# Autodesk Inventor assembly: kitchen
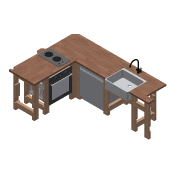
[picture p0: Inventor's stored thumbnail of the model, 180x180]
Saved by Autodesk Inventor 2018 (Build 220112000, 112)
## iProperties
Created: 2017-12-11
Part Number: kitchen
Document SubType Name: Assembly
Designer: sawaiz
Author: sawaiz
## Documents named in this file (12)
- C:\Users\sawaiz\OneDrive\personal\berlin\Move\larkspur\kitchen\kitchen.iam
- C:\Users\sawaiz\OneDrive\personal\berlin\Move\larkspur\kitchen\countertopSink.ipt
- C:\Users\sawaiz\OneDrive\personal\berlin\Move\larkspur\kitchen\Sink 63220001.ipt
- C:\Users\sawaiz\OneDrive\personal\berlin\Move\larkspur\kitchen\mieleWT946.ipt
- C:\Users\sawaiz\OneDrive\personal\berlin\Move\larkspur\kitchen\frameVertical.ipt
- C:\Users\sawaiz\OneDrive\personal\berlin\Move\larkspur\kitchen\frameSides.iam
- C:\Users\sawaiz\OneDrive\personal\berlin\Move\larkspur\kitchen\stoveCountertop.ipt
- C:\Users\sawaiz\OneDrive\personal\berlin\Move\larkspur\kitchen\Samsung BF641FGB.ipt
- C:\Users\sawaiz\OneDrive\personal\berlin\Move\larkspur\kitchen\Cooktop.ipt
- C:\Users\sawaiz\OneDrive\personal\berlin\Move\larkspur\kitchen\sink mixture DND assembly - sink mixture DND-1.ipt
- C:\Users\sawaiz\OneDrive\personal\berlin\Move\larkspur\kitchen\horizontalUnderSink.ipt
- C:\Users\sawaiz\OneDrive\personal\berlin\Move\larkspur\kitchen\kitchen.xlsx
## Components (15 placed, 10 different names)
1. countertopSink:1 — Flush:1, Mate:1, Mate:2, Mate:3, Flush:3, Mate:7, Flush:15, Mate:8, Flush:23, Flush:24, Mate:12, Flush:26, Mate:13, Flush:34, Mate:14, Mate:25
2. Sink 63220001:1 — Flush:1, Mate:1, Mate:2
3. mieleWT946:1 — Mate:3, Flush:3, Flush:16, Mate:9, Flush:33
4. frameVertical:5 — Mate:7, Flush:15, Flush:25
5. frameSides:1 [sub-assembly] — Flush:17, Flush:20, Flush:23, Flush:25
6. frameSides:2 [sub-assembly] — Flush:16, Flush:17, Flush:21, Mate:9, Flush:24, Flush:38, Flush:39
7. frameSides:4 [sub-assembly] — Flush:20, Flush:21, Mate:8, Mate:11, Angle:1, Flush:33
8. frameSides:5 [sub-assembly] — Mate:11, Angle:1, Mate:12, Flush:26, Mate:20, Flush:35
9. frameSides:7 [sub-assembly] — Mate:18, Mate:21, Mate:22, Mate:23, Flush:35, Flush:36
10. stoveCountertop:1 — Mate:13, Flush:34, Mate:14, Mate:19, Angle:2, Mate:23, Mate:24, Flush:37
11. Samsung BF641FGB:1 — Mate:18, Mate:20, Mate:21, Mate:22
12. Cooktop:1 — Mate:19, Angle:2
13. frameSides:8 [sub-assembly] — Flush:36, Mate:24, Flush:37
14. sink mixture DND assembly - sink mixture DND-1:1 — Mate:25
15. horizontalUnderSink:1 — Flush:38, Flush:39
## Relationships (38: Flush 18, Mate 18, Angle 2)
- Flush:1: countertopSink:1 ↔ Sink 63220001:1
- Mate:1: countertopSink:1 ↔ Sink 63220001:1
- Mate:2 (2.5 mm): countertopSink:1 ↔ Sink 63220001:1
- Mate:3: countertopSink:1 ↔ mieleWT946:1
- Flush:3 (50 mm): countertopSink:1 ↔ mieleWT946:1
- Mate:7: countertopSink:1 ↔ frameVertical:5
- Flush:15 (50 mm): countertopSink:1 ↔ frameVertical:5
- Flush:16: mieleWT946:1 ↔ frameSides:2
- Flush:17: frameSides:1 ↔ frameSides:2
- Flush:20: frameSides:1 ↔ frameSides:4
- Flush:21: frameSides:2 ↔ frameSides:4
- Mate:8: countertopSink:1 ↔ frameSides:4
- Mate:9 (2.5 mm): mieleWT946:1 ↔ frameSides:2
- Flush:23: countertopSink:1 ↔ frameSides:1
- Flush:24: countertopSink:1 ↔ frameSides:2
- Mate:11: frameSides:4 ↔ frameSides:5
- Angle:1 (270 deg): frameSides:4 ↔ frameSides:5
- Mate:12: countertopSink:1 ↔ frameSides:5
- Flush:25: frameVertical:5 ↔ frameSides:1
- Flush:26 (50 mm): countertopSink:1 ↔ frameSides:5
- Flush:33: mieleWT946:1 ↔ frameSides:4
- Mate:13: countertopSink:1 ↔ stoveCountertop:1
- Flush:34: countertopSink:1 ↔ stoveCountertop:1
- Mate:14: countertopSink:1 ↔ stoveCountertop:1
- Mate:18: frameSides:7 ↔ Samsung BF641FGB:1
- Mate:19: stoveCountertop:1 ↔ Cooktop:1
- Angle:2 (0 deg): stoveCountertop:1 ↔ Cooktop:1
- Mate:20: frameSides:5 ↔ Samsung BF641FGB:1
- Mate:21: frameSides:7 ↔ Samsung BF641FGB:1
- Mate:22: frameSides:7 ↔ Samsung BF641FGB:1
- Mate:23: frameSides:7 ↔ stoveCountertop:1
- Flush:35: frameSides:5 ↔ frameSides:7
- Flush:36: frameSides:7 ↔ frameSides:8
- Mate:24: stoveCountertop:1 ↔ frameSides:8
- Flush:37 (50 mm): stoveCountertop:1 ↔ frameSides:8
- Mate:25: countertopSink:1 ↔ sink mixture DND assembly - sink mixture DND-1:1
- Flush:38: frameSides:2 ↔ horizontalUnderSink:1
- Flush:39: frameSides:2 ↔ horizontalUnderSink:1
## Named parameters: lumberWidth = 58 mm, lumberDepth = 108 mm, counterThickness = 38 mm, frameHeight = 820 mm, counterHeight = 858 mm, counterDepth = 635 mm, frameOverhang = 50 mm
